# Autodesk Inventor assembly: cadena conjunto
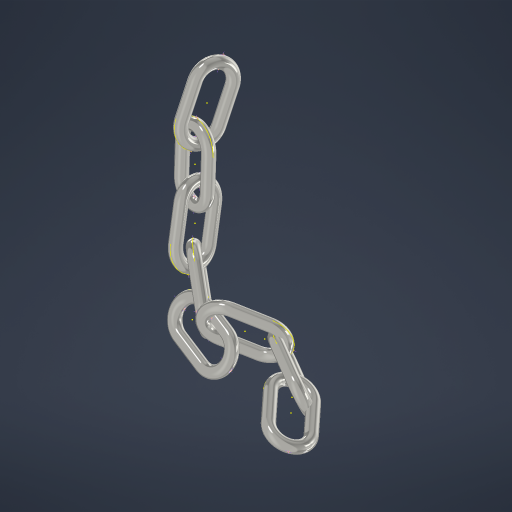
[picture p0: Inventor's stored thumbnail of the model, 512x512]
Saved by Autodesk Inventor 2024 (Build 280153000, 153)
## iProperties
Created: 2015-11-26
Part Number: cadena conjunto
Document SubType Name: Assembly
Designer: H. Valenzuela B.
Author: H. Valenzuela B.
## Documents named in this file (2)
- C:\Users\javie\Downloads\cadena-chain-2.snapshot.2\cadena.iam
- C:\Users\javie\Downloads\cadena-chain-2.snapshot.2\cadena.ipt
## Components (8 placed, 1 different names)
1. cadena:5
2. cadena:8
3. cadena:9
4. cadena:13
5. cadena:15
6. cadena:16
7. cadena:17
8. cadena:18
## Relationships (4: Tangent 4)
- [Tangent]: cadena:8 ↔ cadena:9
- [Tangent]: cadena:15 ↔ cadena:16
- [Tangent]: cadena:17 ↔ cadena:18
- [Tangent]: cadena:16 ↔ cadena:17
## Named parameters: d8_d2 = 0 mm, d12_d6_d3_d2 = 0 mm, d13_d7_d4 = 0 mm, d14_d8_d2 = 0 mm
